# Autodesk Inventor assembly: A2017_T2_06
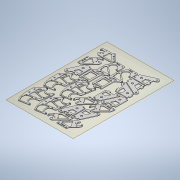
[picture p0: Inventor's stored thumbnail of the model, 180x180]
Saved by Autodesk Inventor 2020 (Build 240168000, 168)
## iProperties
Created: 2021-08-27
Part Number: A2017_T2_06
Document SubType Name: Assembly
Designer: Masato
Author: Masato
## Documents named in this file (6)
- C:\Users\naoki\Documents\Inventor\CitBrains\git_clone\SUSTAINA_ver1_0\A_T2_175\SUSTAINA-OP\Cam\A2017_T2_06.iam
- C:\Users\naoki\Documents\Inventor\CitBrains\git_clone\SUSTAINA_ver1_0\A_T2_175\SUSTAINA-OP\Cam\DisposableBoard.ipt
- C:\Users\naoki\Documents\Inventor\CitBrains\git_clone\SUSTAINA_ver1_0\A_T2_175\SUSTAINA-OP\LowerBody\Knee\Knee_side_frame.ipt
- C:\Users\naoki\Documents\Inventor\CitBrains\git_clone\SUSTAINA_ver1_0\A_T2_175\SUSTAINA-OP\LowerBody\Leg_joint\Leg_joint_pitch_frame.ipt
- C:\Users\naoki\Documents\Inventor\CitBrains\git_clone\SUSTAINA_ver1_0\A_T2_175\SUSTAINA-OP\UpperBody\Arm\Shoulder_side_frame.ipt
- C:\Users\naoki\Documents\Inventor\CitBrains\git_clone\SUSTAINA_ver1_0\A_T2_175\SUSTAINA-OP\LowerBody\Ankle\Ankle_side_frame.ipt
## Components (21 placed, 5 different names)
1. DisposableBoard:1 — メイト:2, メイト:1, フラッシュ:1, フラッシュ:2, 正接:1, フラッシュ:3, メイト:4, メイト:7, メイト:8, メイト:9, メイト:10, フラッシュ:4, フラッシュ:5, メイト:19, メイト:20, メイト:21, メイト:22, メイト:26, メイト:27, メイト:28, メイト:29, メイト:30, メイト:31, メイト:32, メイト:33, 正接:6, 角度:1, フラッシュ:7, 正接:8, 角度:2, 角度:3
2. Leg_joint_pitch_frame:1 — メイト:10, メイト:14, メイト:15, 正接:2, フラッシュ:6, メイト:24
3. Leg_joint_pitch_frame:2 — メイト:9, メイト:13, メイト:14, フラッシュ:6, メイト:23
4. Shoulder_side_frame:2 — メイト:7, フラッシュ:4, メイト:11, メイト:13
5. Shoulder_side_frame:1 — メイト:8, メイト:11, フラッシュ:5, メイト:15
6. Shoulder_side_frame:3 — メイト:17, メイト:18, メイト:20, メイト:24, 正接:4
7. Shoulder_side_frame:4 — メイト:18, メイト:19, メイト:23, メイト:25
8. Leg_joint_pitch_frame:3 — 正接:3, メイト:16, メイト:17, メイト:21
9. Leg_joint_pitch_frame:4 — 正接:3, メイト:16, メイト:22, メイト:25, メイト:36
10. Shoulder_side_frame:6 — メイト:26, 正接:7, 正接:8, 角度:2, メイト:35
11. Shoulder_side_frame:7 — メイト:27, フラッシュ:7, メイト:34, 正接:7
12. Leg_joint_pitch_frame:5 — メイト:29, 正接:5, 正接:6, 角度:1, メイト:34
13. Leg_joint_pitch_frame:6 — メイト:31, メイト:36, メイト:37, 正接:12
14. Leg_joint_pitch_frame:7 — メイト:32, メイト:37, メイト:38, メイト:39
15. Leg_joint_pitch_frame:8 — メイト:33, メイト:38, メイト:40
16. Ankle_side_frame:1 — メイト:30, 角度:4, 正接:10, 正接:11, メイト:39, メイト:40, 正接:12
17. Ankle_side_frame:2 — メイト:28, 角度:3, 角度:4, メイト:35, 正接:9, 正接:11
18. Knee_side_frame:1 — 正接:1, フラッシュ:3, メイト:4
19. Knee_side_frame:3 — 正接:5, 正接:9
20. Knee_side_frame:4 — 正接:2
21. Knee_side_frame:5 — 正接:4, 正接:10
## Component patterns: (4 elements, first: Knee_side_frame:1)
## Relationships (59: Mate 36, Tangent 12, Flush 7, Angle 4)
- メイト:2 [Mate]: DisposableBoard:1
- メイト:1 [Mate]: DisposableBoard:1
- フラッシュ:1 [Flush]: DisposableBoard:1
- フラッシュ:2 [Flush]: DisposableBoard:1
- 正接:1 [Tangent] (2.5 mm): DisposableBoard:1 ↔ Knee_side_frame:1
- フラッシュ:3 [Flush] (2 mm): DisposableBoard:1 ↔ Knee_side_frame:1
- メイト:4 [Mate]: DisposableBoard:1 ↔ Knee_side_frame:1
- メイト:7 [Mate]: DisposableBoard:1 ↔ Shoulder_side_frame:2
- メイト:8 [Mate]: DisposableBoard:1 ↔ Shoulder_side_frame:1
- メイト:9 [Mate]: DisposableBoard:1 ↔ Leg_joint_pitch_frame:2
- メイト:10 [Mate]: DisposableBoard:1 ↔ Leg_joint_pitch_frame:1
- フラッシュ:4 [Flush] (2 mm): DisposableBoard:1 ↔ Shoulder_side_frame:2
- メイト:11 [Mate] (2.5 mm): Shoulder_side_frame:2 ↔ Shoulder_side_frame:1
- メイト:13 [Mate] (2.5 mm): Leg_joint_pitch_frame:2 ↔ Shoulder_side_frame:2
- メイト:14 [Mate] (2.5 mm): Leg_joint_pitch_frame:1 ↔ Leg_joint_pitch_frame:2
- フラッシュ:5 [Flush] (2 mm): DisposableBoard:1 ↔ Shoulder_side_frame:1
- メイト:15 [Mate] (2.5 mm): Leg_joint_pitch_frame:1 ↔ Shoulder_side_frame:1
- 正接:2 [Tangent] (2.5 mm): Leg_joint_pitch_frame:1 ↔ Knee_side_frame:4
- フラッシュ:6 [Flush]: Leg_joint_pitch_frame:1 ↔ Leg_joint_pitch_frame:2
- 正接:3 [Tangent]: Leg_joint_pitch_frame:3 ↔ Leg_joint_pitch_frame:4
- メイト:16 [Mate] (2.5 mm): Leg_joint_pitch_frame:3 ↔ Leg_joint_pitch_frame:4
- メイト:17 [Mate] (2.5 mm): Shoulder_side_frame:3 ↔ Leg_joint_pitch_frame:3
- メイト:18 [Mate] (2.5 mm): Shoulder_side_frame:3 ↔ Shoulder_side_frame:4
- メイト:19 [Mate]: DisposableBoard:1 ↔ Shoulder_side_frame:4
- メイト:20 [Mate]: DisposableBoard:1 ↔ Shoulder_side_frame:3
- メイト:21 [Mate]: DisposableBoard:1 ↔ Leg_joint_pitch_frame:3
- メイト:22 [Mate]: DisposableBoard:1 ↔ Leg_joint_pitch_frame:4
- メイト:23 [Mate] (2.5 mm): Leg_joint_pitch_frame:2 ↔ Shoulder_side_frame:4
- メイト:24 [Mate] (2.5 mm): Leg_joint_pitch_frame:1 ↔ Shoulder_side_frame:3
- 正接:4 [Tangent] (2.5 mm): Shoulder_side_frame:3 ↔ Knee_side_frame:5
- メイト:25 [Mate] (2.5 mm): Shoulder_side_frame:4 ↔ Leg_joint_pitch_frame:4
- メイト:26 [Mate]: DisposableBoard:1 ↔ Shoulder_side_frame:6
- メイト:27 [Mate]: DisposableBoard:1 ↔ Shoulder_side_frame:7
- メイト:28 [Mate]: DisposableBoard:1 ↔ Ankle_side_frame:2
- メイト:29 [Mate]: DisposableBoard:1 ↔ Leg_joint_pitch_frame:5
- メイト:30 [Mate]: DisposableBoard:1 ↔ Ankle_side_frame:1
- メイト:31 [Mate]: DisposableBoard:1 ↔ Leg_joint_pitch_frame:6
- メイト:32 [Mate]: DisposableBoard:1 ↔ Leg_joint_pitch_frame:7
- メイト:33 [Mate]: DisposableBoard:1 ↔ Leg_joint_pitch_frame:8
- 正接:5 [Tangent] (2.5 mm): Leg_joint_pitch_frame:5 ↔ Knee_side_frame:3
- 正接:6 [Tangent] (2 mm): DisposableBoard:1 ↔ Leg_joint_pitch_frame:5
- 角度:1 [Angle] (180 deg): DisposableBoard:1 ↔ Leg_joint_pitch_frame:5
- フラッシュ:7 [Flush] (2 mm): DisposableBoard:1 ↔ Shoulder_side_frame:7
- メイト:34 [Mate] (2.5 mm): Shoulder_side_frame:7 ↔ Leg_joint_pitch_frame:5
- 正接:7 [Tangent] (2.5 mm): Shoulder_side_frame:6 ↔ Shoulder_side_frame:7
- 正接:8 [Tangent] (2.5 mm): DisposableBoard:1 ↔ Shoulder_side_frame:6
- 角度:2 [Angle] (0 deg): DisposableBoard:1 ↔ Shoulder_side_frame:6
- 角度:3 [Angle] (0 deg): DisposableBoard:1 ↔ Ankle_side_frame:2
- 角度:4 [Angle] (0 deg): Ankle_side_frame:1 ↔ Ankle_side_frame:2
- メイト:35 [Mate] (2.5 mm): Shoulder_side_frame:6 ↔ Ankle_side_frame:2
- 正接:9 [Tangent] (2.5 mm): Ankle_side_frame:2 ↔ Knee_side_frame:3
- 正接:10 [Tangent] (2.5 mm): Ankle_side_frame:1 ↔ Knee_side_frame:5
- 正接:11 [Tangent] (2.5 mm): Ankle_side_frame:1 ↔ Ankle_side_frame:2
- メイト:36 [Mate] (2.5 mm): Leg_joint_pitch_frame:4 ↔ Leg_joint_pitch_frame:6
- メイト:37 [Mate] (2.5 mm): Leg_joint_pitch_frame:6 ↔ Leg_joint_pitch_frame:7
- メイト:38 [Mate] (2.5 mm): Leg_joint_pitch_frame:7 ↔ Leg_joint_pitch_frame:8
- メイト:39 [Mate] (2.5 mm): Leg_joint_pitch_frame:7 ↔ Ankle_side_frame:1
- メイト:40 [Mate] (2.5 mm): Leg_joint_pitch_frame:8 ↔ Ankle_side_frame:1
- 正接:12 [Tangent] (2.5 mm): Leg_joint_pitch_frame:6 ↔ Ankle_side_frame:1
